# Autodesk Inventor assembly: side of drivetrain
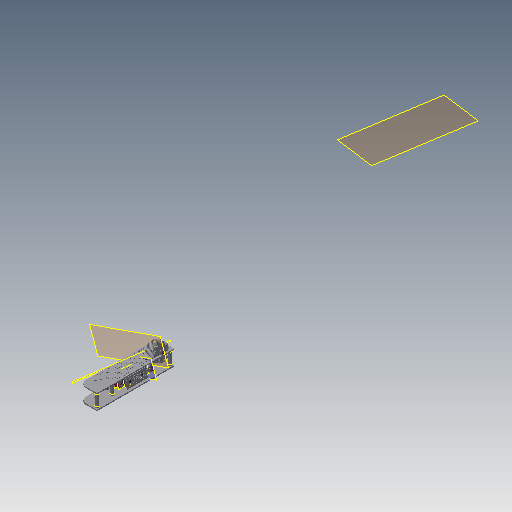
[picture p0: Inventor's stored thumbnail of the model, 512x512]
Saved by Autodesk Inventor 2020 (Build 240168000, 168)
## iProperties
Created: 2019-10-04
Part Number: side of drivetrain
Document SubType Name: Assembly
Designer: ball
Author: ball
## Documents named in this file (14)
- C:\FTC\FTC8863CAD\2019 Robot\Mecanum Drive Train\side of drivetrain.iam
- C:\FTC\FTC8863CAD\2019 Robot\Mecanum Drive Train\wheel with drive motor top.iam
- C:\FTC\FTC8863CAD\2019 Robot\Mecanum Drive Train\wheel with drive motor floor.iam
- C:\FTC\FTC8863CAD\2019 Robot\Mecanum Drive Train\inside wall.ipt
- C:\FTC\FTC8863CAD\2019 Robot\Mecanum Drive Train\center motor mount.ipt
- C:\FTC\FTC8863CAD\2019 Robot\Mecanum Drive Train\outside wall.ipt
- C:\FTC\FTC8863CAD\2019 Robot\Mecanum Drive Train\motor mount cap.ipt
- C:\FTC\FTC8863CAD\2019 Robot\Odoemetry module\OdometryAssembly.iam
- C:\FTC\FTC8863CAD\2019 Robot\Mecanum Drive Train\standoff for walls.ipt
- C:\FTC\FTC8863CAD\StepLibraries\Screws\M4 x 100 SOCKET HEAD CAP SCREW.ipt
- C:\FTC\FTC8863CAD\StepLibraries\Nuts\M4 NYLON-INSERT LOCKNUT.ipt
- C:\FTC\FTC8863CAD\Actobotics\633 parts\633104.ipt
- C:\FTC\FTC8863CAD\2019 Robot\Odoemetry module\m4 x 1_316 spacer.ipt
- C:\FTC\FTC8863CAD\StepLibraries\Nuts\6-32 NYLON-INSERT LOCKNUT.ipt
## Components (17 placed, 13 different names)
1. wheel with drive motor top:1 [sub-assembly] — Flush:4, Mate:5, Flush:6, Mate:7, Mate:8, Mate:12, Mate:14
2. wheel with drive motor floor:1 [sub-assembly] — Flush:4, Mate:5, Flush:6, Mate:9, Mate:13
3. inside wall — Mate:7, Mate:8, Mate:9, Mate:11, Mate:23, Mate:24, Angle:3, Mate:25, Mate:26, Angle:4, Mate:29, Mate:35
4. center motor mount:1 — Flush:7, Flush:8, Mate:17, Mate:18, Mate:37, Mate:38, Mate:39, Mate:40
5. outside wall:1 — Mate:12, Mate:13, Mate:14, Angle:1, Mate:21, Mate:22, Angle:2, Mate:27, Mate:28, Mate:33
6. motor mount cap:1 — Flush:7, Mate:18
7. motor mount cap:2 — Flush:8, Mate:17
8. OdometryAssembly:1 [sub-assembly] — Angle:1, Mate:31, Mate:34
9. standoff for walls:1 — Mate:21, Mate:22, Angle:2
10. standoff for walls:2 — Mate:23, Mate:24, Angle:3
11. standoff for walls:3 — Mate:25, Mate:26, Angle:4
12. M4 x 100 SOCKET HEAD CAP SCREW:1 — Mate:27, Mate:28, Mate:30, Mate:31, Mate:32, Mate:36
13. M4 NYLON-INSERT LOCKNUT:1 — Mate:29, Mate:30
14. 633104:1 — Mate:32, Mate:33, Mate:34
15. m4 x 1_316 spacer:1 — Mate:35, Mate:36
16. 6-32 NYLON-INSERT LOCKNUT:1 — Mate:37, Mate:38
17. 6-32 NYLON-INSERT LOCKNUT:2 — Mate:39, Mate:40
## Relationships (38: Mate 30, Flush 4, Angle 4)
- Flush:4: wheel with drive motor top:1 ↔ wheel with drive motor floor:1
- Mate:5 (44.3484 mm): wheel with drive motor top:1 ↔ wheel with drive motor floor:1
- Flush:6 (330.2 mm): wheel with drive motor top:1 ↔ wheel with drive motor floor:1
- Mate:7: wheel with drive motor top:1 ↔ inside wall
- Mate:8: wheel with drive motor top:1 ↔ inside wall
- Mate:9: wheel with drive motor floor:1 ↔ inside wall
- Mate:11: inside wall
- Mate:12: wheel with drive motor top:1 ↔ outside wall:1
- Mate:13: wheel with drive motor floor:1 ↔ outside wall:1
- Mate:14: wheel with drive motor top:1 ↔ outside wall:1
- Flush:7: center motor mount:1 ↔ motor mount cap:1
- Flush:8: center motor mount:1 ↔ motor mount cap:2
- Mate:17: center motor mount:1 ↔ motor mount cap:2
- Mate:18: center motor mount:1 ↔ motor mount cap:1
- Angle:1 (-10 deg): outside wall:1 ↔ OdometryAssembly:1
- Mate:21: outside wall:1 ↔ standoff for walls:1
- Mate:22: outside wall:1 ↔ standoff for walls:1
- Angle:2 (0 deg): outside wall:1 ↔ standoff for walls:1
- Mate:23: inside wall ↔ standoff for walls:2
- Mate:24: inside wall ↔ standoff for walls:2
- Angle:3 (0 deg): inside wall ↔ standoff for walls:2
- Mate:25: inside wall ↔ standoff for walls:3
- Mate:26: inside wall ↔ standoff for walls:3
- Angle:4 (0 deg): inside wall ↔ standoff for walls:3
- Mate:27: outside wall:1 ↔ M4 x 100 SOCKET HEAD CAP SCREW:1
- Mate:28: outside wall:1 ↔ M4 x 100 SOCKET HEAD CAP SCREW:1
- Mate:29: inside wall ↔ M4 NYLON-INSERT LOCKNUT:1
- Mate:30: M4 x 100 SOCKET HEAD CAP SCREW:1 ↔ M4 NYLON-INSERT LOCKNUT:1
- Mate:31: OdometryAssembly:1 ↔ M4 x 100 SOCKET HEAD CAP SCREW:1
- Mate:32: M4 x 100 SOCKET HEAD CAP SCREW:1 ↔ 633104:1
- Mate:33: outside wall:1 ↔ 633104:1
- Mate:34: OdometryAssembly:1 ↔ 633104:1
- Mate:35: inside wall ↔ m4 x 1_316 spacer:1
- Mate:36: M4 x 100 SOCKET HEAD CAP SCREW:1 ↔ m4 x 1_316 spacer:1
- Mate:37: center motor mount:1 ↔ 6-32 NYLON-INSERT LOCKNUT:1
- Mate:38: center motor mount:1 ↔ 6-32 NYLON-INSERT LOCKNUT:1
- Mate:39: center motor mount:1 ↔ 6-32 NYLON-INSERT LOCKNUT:2
- Mate:40: center motor mount:1 ↔ 6-32 NYLON-INSERT LOCKNUT:2
